# Autodesk Inventor assembly: Right Drive Wheel Assembly
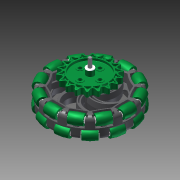
[picture p0: Inventor's stored thumbnail of the model, 180x180]
Saved by Autodesk Inventor 2012 (Build 160160000, 160)
## iProperties
Created: 2011-09-10
Part Number: Right Drive Wheel Assembly
Document SubType Name: Assembly
Designer: Wade
Author: Wade
## Documents named in this file (7)
- C:\Users\Wade\Documents\1103 Robot - CAD Assembly\Right Drive Wheel Assembly.iam
- C:\Users\Wade\Documents\1103 Robot - CAD Assembly\18 Tooth HS Sprocket.ipt
- C:\Users\Wade\Documents\24C VEX CAD Files\Wheels\4'' Omni-Directional Wheel.iam
- C:\Users\Wade\Documents\24C VEX CAD Files\Washers & Spacers\Spacer (Nylon), 0.500''.ipt
- C:\Users\Wade\Documents\24C VEX CAD Files\Washers & Spacers\Washer, Delrin.ipt
- C:\Users\Wade\Documents\24C VEX CAD Files\Other Parts\Shaft Collar (with Set Screw Installed).ipt
- C:\Users\Wade\Documents\1103 Robot - CAD Assembly\1103 custom.ipt
## Components (6 placed, 6 different names)
1. 18 Tooth HS Sprocket:1 — Flush:1, Flush:3, Mate:6, Mate:10, Mate:11, Mate:12, Mate:13
2. 4'' Omni-Directional Wheel:1 [sub-assembly] — Mate:1, Flush:1, Mate:3, Flush:2, Flush:3, Mate:8, Mate:9
3. Spacer (Nylon), 0.500'':1 — Mate:1, Mate:9, Flush:4
4. Washer, Delrin:1 — Mate:6, Mate:11
5. Shaft Collar (with Set Screw Installed):1 — Mate:3, Flush:2, Mate:8, Mate:10
6. 1103 custom:1 — Mate:12, Mate:13, Flush:4
## Relationships (13: Mate 9, Flush 4)
- Mate:1: 4'' Omni-Directional Wheel:1 ↔ Spacer (Nylon), 0.500'':1
- Flush:1: 18 Tooth HS Sprocket:1 ↔ 4'' Omni-Directional Wheel:1
- Mate:3: 4'' Omni-Directional Wheel:1 ↔ Shaft Collar (with Set Screw Installed):1
- Flush:2: 4'' Omni-Directional Wheel:1 ↔ Shaft Collar (with Set Screw Installed):1
- Flush:3: 18 Tooth HS Sprocket:1 ↔ 4'' Omni-Directional Wheel:1
- Mate:6: 18 Tooth HS Sprocket:1 ↔ Washer, Delrin:1
- Mate:8: 4'' Omni-Directional Wheel:1 ↔ Shaft Collar (with Set Screw Installed):1
- Mate:9: 4'' Omni-Directional Wheel:1 ↔ Spacer (Nylon), 0.500'':1
- Mate:10: 18 Tooth HS Sprocket:1 ↔ Shaft Collar (with Set Screw Installed):1
- Mate:11: 18 Tooth HS Sprocket:1 ↔ Washer, Delrin:1
- Mate:12: 18 Tooth HS Sprocket:1 ↔ 1103 custom:1
- Mate:13: 18 Tooth HS Sprocket:1 ↔ 1103 custom:1
- Flush:4 (-6.35 mm): Spacer (Nylon), 0.500'':1 ↔ 1103 custom:1
